# Autodesk Inventor assembly: Aero_assembly
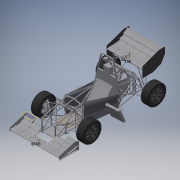
[picture p0: Inventor's stored thumbnail of the model, 180x180]
Saved by Autodesk Inventor 2018.2 (Build 222227000, 227)
## iProperties
Created: 2018-03-12
Part Number: Aero_assembly
Material: 一般
Document SubType Name: Assembly
Designer: ku_sk
Author: ku_sk
## Documents named in this file (20)
- Z:\各班フォルダ\2018\ボディ\エアロ\Aero\KS-15\Aero_assembly.iam
- Z:\各班フォルダ\2018\ボディ\エアロ\Aero\KS-15\Fr.wing\Fr.wing_assy.iam
- Z:\各班フォルダ\2018\ボディ\エアロ\Aero\KS-15\Rr.wing\Rr.wing_assy.iam
- Z:\各班フォルダ\2018\ボディ\エアロ\Aero\KS-15\body\2018 zentai assembly.iam
- Z:\各班フォルダ\2018\ボディ\エアロ\Aero\KS-15\Pontoon\2018 radiator analysis.iam
- Z:\各班フォルダ\2018\ボディ\エアロ\Aero\KS-15\body\parts\2015Wheel watanabe.ipt
- Z:\各班フォルダ\2018\ボディ\エアロ\Aero\KS-15\Rr.wing\parts\stay\end\parts\Symmetry of POS_8ECBall.ipt
- Z:\各班フォルダ\2018\ボディ\エアロ\Aero\KS-15\Rr.wing\parts\stay\collar_6.2.ipt
- Z:\各班フォルダ\2018\ボディ\エアロ\Aero\KS-15\Rr.wing\parts\stay\collar_4.2.ipt
- Z:\各班フォルダ\2018\ボディ\エアロ\Aero\KS-15\Rr.wing\parts\stay\stay1.iam
- Z:\各班フォルダ\2018\ボディ\エアロ\Aero\KS-15\Rr.wing\parts\stay\end\stay end.iam
- Z:\各班フォルダ\2018\ボディ\エアロ\Aero\KS-15\Rr.wing\parts\stay\stay2.iam
- Z:\各班フォルダ\2018\ボディ\エアロ\Aero\KS-15\Rr.wing\parts\stay\stay3.iam
- Z:\各班フォルダ\2018\ボディ\エアロ\Aero\KS-15\Rr.wing\parts\stay\end\parts\Symmetry of POS_8ECBall_MIR.ipt
- Z:\各班フォルダ\2018\ボディ\エアロ\Aero\KS-15\Rr.wing\parts\stay\collar_6.2_MIR.ipt
- Z:\各班フォルダ\2018\ボディ\エアロ\Aero\KS-15\Rr.wing\parts\stay\collar_4.2_MIR.ipt
- Z:\各班フォルダ\2018\ボディ\エアロ\Aero\KS-15\Rr.wing\parts\stay\stay1_MIR.iam
- Z:\各班フォルダ\2018\ボディ\エアロ\Aero\KS-15\Rr.wing\parts\stay\end\stay end_MIR.iam
- Z:\各班フォルダ\2018\ボディ\エアロ\Aero\KS-15\Rr.wing\parts\stay\stay2_MIR.iam
- Z:\各班フォルダ\2018\ボディ\エアロ\Aero\KS-15\Rr.wing\parts\stay\stay3_MIR.iam
## Components (36 placed, 19 different names)
1. 2018 zentai assembly:1 [sub-assembly] — メイト:8, メイト:9, メイト:10, メイト:14, メイト:15, フラッシュ:9, フラッシュ:10, メイト:18, メイト:19, メイト:20, メイト:21, メイト:22, メイト:23, メイト:28, メイト:29, メイト:30, メイト:31
2. 2018 radiator analysis:1 [sub-assembly] — メイト:11, メイト:12, メイト:13
3. Fr.wing_assy:1 [sub-assembly] — フラッシュ:1
4. Rr.wing_assy:1 [sub-assembly] — フラッシュ:6, フラッシュ:7, フラッシュ:8, ボール:1, ボール:3, ボール:6
5. 2015Wheel watanabe:1 — メイト:14, フラッシュ:10
6. 2015Wheel watanabe:2 — メイト:15, フラッシュ:9
7. Symmetry of POS_8ECBall:1 — メイト:24, メイト:25, ボール:2
8. Symmetry of POS_8ECBall:2 — メイト:26, メイト:27, ボール:4
9. collar_6.2:1 — メイト:16, メイト:18, メイト:19, メイト:25
10. collar_6.2:2 — メイト:16, メイト:22, メイト:24
11. collar_6.2:3 — メイト:17, メイト:23, メイト:26
12. collar_6.2:4 — メイト:17, メイト:20, メイト:21, メイト:27
13. collar_4.2:1 — メイト:28, メイト:30, メイト:32
14. collar_4.2:2 — メイト:29, メイト:31, メイト:33
15. Symmetry of POS_8ECBall:3 — メイト:32, メイト:33, ボール:5
16. stay1:1 [sub-assembly] — ボール:1, メイト:34
17. stay end:1 [sub-assembly] — ボール:2, メイト:34
18. stay2:1 [sub-assembly] — ボール:3, メイト:35
19. stay end:2 [sub-assembly] — ボール:4, メイト:35
20. stay end:3 [sub-assembly] — ボール:6, メイト:36
21. stay3:1 [sub-assembly] — ボール:5, メイト:36
22. Symmetry of POS_8ECBall_MIR:1 — メイト:37, メイト:38, ボール:7
23. Symmetry of POS_8ECBall_MIR:2 — メイト:40, メイト:41, ボール:8
24. collar_6.2_MIR:1 — メイト:37, メイト:39
25. collar_6.2_MIR:2 — メイト:38, メイト:39
26. collar_6.2_MIR:3 — メイト:40, メイト:42
27. collar_6.2_MIR:4 — メイト:41, メイト:42
28. collar_4.2_MIR:1 — メイト:44
29. collar_4.2_MIR:2 — メイト:43
30. Symmetry of POS_8ECBall_MIR:3 — メイト:43, メイト:44, ボール:9
31. stay1_MIR:1 [sub-assembly] — メイト:45
32. stay end_MIR:1 [sub-assembly] — メイト:45, ボール:7
33. stay2_MIR:1 [sub-assembly] — メイト:46
34. stay end_MIR:2 [sub-assembly] — メイト:46, ボール:8
35. stay end_MIR:3 [sub-assembly] — メイト:47
36. stay3_MIR:1 [sub-assembly] — メイト:47, ボール:9
## Relationships (55: Mate 40, BallJoint 9, Flush 6)
- フラッシュ:1 [Flush]: Fr.wing_assy:1
- フラッシュ:6 [Flush]: Rr.wing_assy:1
- フラッシュ:7 [Flush] (460 mm): Rr.wing_assy:1
- メイト:8 [Mate]: 2018 zentai assembly:1
- メイト:9 [Mate]: 2018 zentai assembly:1
- メイト:10 [Mate]: 2018 zentai assembly:1
- メイト:11 [Mate]: 2018 radiator analysis:1
- メイト:12 [Mate]: 2018 radiator analysis:1
- メイト:13 [Mate]: 2018 radiator analysis:1
- フラッシュ:8 [Flush] (-1080 mm): Rr.wing_assy:1
- メイト:14 [Mate]: 2018 zentai assembly:1 ↔ 2015Wheel watanabe:1
- メイト:15 [Mate]: 2018 zentai assembly:1 ↔ 2015Wheel watanabe:2
- フラッシュ:9 [Flush]: 2018 zentai assembly:1 ↔ 2015Wheel watanabe:2
- フラッシュ:10 [Flush]: 2018 zentai assembly:1 ↔ 2015Wheel watanabe:1
- メイト:16 [Mate]: collar_6.2:1 ↔ collar_6.2:2
- メイト:17 [Mate]: collar_6.2:3 ↔ collar_6.2:4
- メイト:18 [Mate]: 2018 zentai assembly:1 ↔ collar_6.2:1
- メイト:19 [Mate]: 2018 zentai assembly:1 ↔ collar_6.2:1
- メイト:20 [Mate]: 2018 zentai assembly:1 ↔ collar_6.2:4
- メイト:21 [Mate]: 2018 zentai assembly:1 ↔ collar_6.2:4
- メイト:22 [Mate]: 2018 zentai assembly:1 ↔ collar_6.2:2
- メイト:23 [Mate]: 2018 zentai assembly:1 ↔ collar_6.2:3
- メイト:24 [Mate]: Symmetry of POS_8ECBall:1 ↔ collar_6.2:2
- メイト:25 [Mate]: Symmetry of POS_8ECBall:1 ↔ collar_6.2:1
- メイト:26 [Mate]: Symmetry of POS_8ECBall:2 ↔ collar_6.2:3
- メイト:27 [Mate]: Symmetry of POS_8ECBall:2 ↔ collar_6.2:4
- メイト:28 [Mate]: 2018 zentai assembly:1 ↔ collar_4.2:1
- メイト:29 [Mate]: 2018 zentai assembly:1 ↔ collar_4.2:2
- メイト:30 [Mate]: 2018 zentai assembly:1 ↔ collar_4.2:1
- メイト:31 [Mate]: 2018 zentai assembly:1 ↔ collar_4.2:2
- メイト:32 [Mate]: collar_4.2:1 ↔ Symmetry of POS_8ECBall:3
- メイト:33 [Mate]: collar_4.2:2 ↔ Symmetry of POS_8ECBall:3
- ボール:1 [BallJoint]: Rr.wing_assy:1 ↔ stay1:1
- ボール:2 [BallJoint]: Symmetry of POS_8ECBall:1 ↔ stay end:1
- メイト:34 [Mate]: stay1:1 ↔ stay end:1
- ボール:3 [BallJoint]: Rr.wing_assy:1 ↔ stay2:1
- ボール:4 [BallJoint]: Symmetry of POS_8ECBall:2 ↔ stay end:2
- メイト:35 [Mate]: stay2:1 ↔ stay end:2
- ボール:5 [BallJoint]: Symmetry of POS_8ECBall:3 ↔ stay3:1
- ボール:6 [BallJoint]: Rr.wing_assy:1 ↔ stay end:3
- メイト:36 [Mate]: stay end:3 ↔ stay3:1
- メイト:37 [Mate]: Symmetry of POS_8ECBall_MIR:1 ↔ collar_6.2_MIR:1
- メイト:38 [Mate]: Symmetry of POS_8ECBall_MIR:1 ↔ collar_6.2_MIR:2
- メイト:39 [Mate]: collar_6.2_MIR:1 ↔ collar_6.2_MIR:2
- メイト:40 [Mate]: Symmetry of POS_8ECBall_MIR:2 ↔ collar_6.2_MIR:3
- メイト:41 [Mate]: Symmetry of POS_8ECBall_MIR:2 ↔ collar_6.2_MIR:4
- メイト:42 [Mate]: collar_6.2_MIR:3 ↔ collar_6.2_MIR:4
- メイト:43 [Mate]: collar_4.2_MIR:2 ↔ Symmetry of POS_8ECBall_MIR:3
- メイト:44 [Mate]: collar_4.2_MIR:1 ↔ Symmetry of POS_8ECBall_MIR:3
- メイト:45 [Mate]: stay1_MIR:1 ↔ stay end_MIR:1
- メイト:46 [Mate]: stay2_MIR:1 ↔ stay end_MIR:2
- メイト:47 [Mate]: stay end_MIR:3 ↔ stay3_MIR:1
- ボール:7 [BallJoint]: Symmetry of POS_8ECBall_MIR:1 ↔ stay end_MIR:1
- ボール:8 [BallJoint]: Symmetry of POS_8ECBall_MIR:2 ↔ stay end_MIR:2
- ボール:9 [BallJoint]: Symmetry of POS_8ECBall_MIR:3 ↔ stay3_MIR:1
